# Autodesk Inventor assembly: KOGANEI_unkown_35
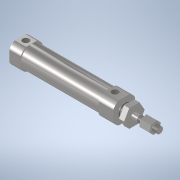
[picture p0: Inventor's stored thumbnail of the model, 180x180]
Saved by Autodesk Inventor 2022.3 (Build 263350000, 350)
## iProperties
Created: 2022-04-18
Part Number: KOGANEI_unkown_35
Document SubType Name: Assembly
Designer: YusukeKunita
Author: YusukeKunita
## Documents named in this file (5)
- C:\Users\YusukeKunita\Documents\GrabCAD\NHK2022\BasicParts\AirCylinder\KOGANEI_unkown_35\KOGANEI_unkown_35.iam
- C:\Users\YusukeKunita\Documents\GrabCAD\NHK2022\BasicParts\AirCylinder\KOGANEI_unkown_35\KOGANEI_unkown_35_main.ipt
- C:\Users\YusukeKunita\Documents\GrabCAD\NHK2022\BasicParts\AirCylinder\KOGANEI_unkown_35\KOGANEI_unkown_35_rod.ipt
- C:\Users\YusukeKunita\Documents\GrabCAD\NHK2022\BasicParts\AirCylinder\KOGANEI_unkown_35\KOGANEI_unkown_35_M10Nut.ipt
- C:\Users\YusukeKunita\Documents\GrabCAD\NHK2022\BasicParts\AirCylinder\KOGANEI_unkown_35\KOGANEI_unkown_35_M5Nut.ipt
## Components (5 placed, 4 different names)
1. KOGANEI_unkown_35_main:1 — 円柱状:1, フラッシュ:1, 回転:1
2. KOGANEI_unkown_35_rod:1 — 円柱状:1, フラッシュ:1, リジッド:1, リジッド:2
3. KOGANEI_unkown_35_M10Nut:1 — 回転:1
4. KOGANEI_unkown_35_M5Nut:1 — リジッド:1
5. KOGANEI_unkown_35_M5Nut:2 — リジッド:2
## Relationships (5: WeldJoint 2, CylindricalJoint 1, Flush 1, RevoluteJoint 1)
- 円柱状:1 [CylindricalJoint]: KOGANEI_unkown_35_main:1 ↔ KOGANEI_unkown_35_rod:1
- フラッシュ:1 [Flush]: KOGANEI_unkown_35_main:1 ↔ KOGANEI_unkown_35_rod:1
- 回転:1 [RevoluteJoint]: KOGANEI_unkown_35_main:1 ↔ KOGANEI_unkown_35_M10Nut:1
- リジッド:1 [WeldJoint]: KOGANEI_unkown_35_rod:1 ↔ KOGANEI_unkown_35_M5Nut:1
- リジッド:2 [WeldJoint]: KOGANEI_unkown_35_rod:1 ↔ KOGANEI_unkown_35_M5Nut:2
